# Autodesk Inventor assembly: 組合檔
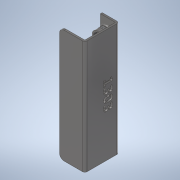
[picture p0: Inventor's stored thumbnail of the model, 180x180]
Saved by Autodesk Inventor 2020 (Build 240168000, 168)
## iProperties
Created: 2015-11-28
Part Number: 組合檔
Document SubType Name: Assembly
Designer: 設計製圖
Author: 設計製圖
## Documents named in this file (5)
- D:\資料庫\設計-3D Project\【May club 】\得利卡-車頂燈架\模型、圖面\短-車頂燈架-組合(#11.02)- 組合件2.iam
- D:\資料庫\設計-3D Project\【 鐵蹄 】\------鐵蹄工廠素材------ -\拉帽-M8.ipt
- D:\資料庫\設計-3D Project\【May club 】\得利卡-車頂燈架\模型、圖面\吊架組件-ㄇ槽(#11.02).ipt
- D:\資料庫\設計-3D Project\【May club 】\得利卡-車頂燈架\模型、圖面\焊接組件-2(#11.02).ipt
- D:\資料庫\設計-3D Project\材料庫\螺帽\白鐵-六角螺帽-M6.ipt
## Components (5 placed, 4 different names)
1. 拉帽-M8:2 — 齊平:6, 貼合:15, 貼合:38
2. 拉帽-M8:1 — 齊平:6, 貼合:15, 貼合:17, 貼合:37
3. 白鐵-六角螺帽-M6:1 — 貼合:44, 貼合:45, 齊平:15
4. 吊架組件-ㄇ槽(#11.02):1 — 貼合:17, 貼合:37, 貼合:38, 貼合:40, 齊平:14, 貼合:41
5. 焊接組件-2(#11.02):1 — 貼合:40, 齊平:14, 貼合:41, 貼合:44, 貼合:45, 齊平:15
## Relationships (11: Mate 8, Flush 3)
- 齊平:6 [Flush]: 拉帽-M8:2 ↔ 拉帽-M8:1
- 貼合:15 [Mate]: 拉帽-M8:2 ↔ 拉帽-M8:1
- 貼合:17 [Mate]: 拉帽-M8:1 ↔ 吊架組件-ㄇ槽(#11.02):1
- 貼合:37 [Mate]: 拉帽-M8:1 ↔ 吊架組件-ㄇ槽(#11.02):1
- 貼合:38 [Mate]: 拉帽-M8:2 ↔ 吊架組件-ㄇ槽(#11.02):1
- 貼合:40 [Mate]: 吊架組件-ㄇ槽(#11.02):1 ↔ 焊接組件-2(#11.02):1
- 齊平:14 [Flush]: 吊架組件-ㄇ槽(#11.02):1 ↔ 焊接組件-2(#11.02):1
- 貼合:41 [Mate]: 吊架組件-ㄇ槽(#11.02):1 ↔ 焊接組件-2(#11.02):1
- 貼合:44 [Mate]: 白鐵-六角螺帽-M6:1 ↔ 焊接組件-2(#11.02):1
- 貼合:45 [Mate]: 白鐵-六角螺帽-M6:1 ↔ 焊接組件-2(#11.02):1
- 齊平:15 [Flush]: 白鐵-六角螺帽-M6:1 ↔ 焊接組件-2(#11.02):1
